# Autodesk Inventor assembly: Ansamblu
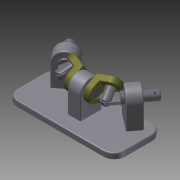
[picture p0: Inventor's stored thumbnail of the model, 180x180]
Saved by Autodesk Inventor 2011 SP2 (Build 150309200, 309)
## iProperties
Created: 2023-03-20
Part Number: Ansamblu
Document SubType Name: Assembly
Designer: utilizator
Author: utilizator
## Documents named in this file (7)
- D:\Studenti\Donisan Enya 1322b\Lab 4\Ansamblu.iam
- D:\Studenti\Donisan Enya 1322b\Lab 4\Placa.ipt
- D:\Studenti\Donisan Enya 1322b\Lab 4\Lagar.ipt
- D:\Studenti\Donisan Enya 1322b\Lab 4\Levier.ipt
- D:\Studenti\Donisan Enya 1322b\Lab 4\Furca.ipt
- D:\Studenti\Donisan Enya 1322b\Lab 4\Arbore.ipt
- D:\Studenti\Donisan Enya 1322b\Lab 4\Ax.ipt
## Components (11 placed, 6 different names)
1. Placa:1 — Mate:1, Mate:2, Mate:3, Mate:4, Mate:5, Angle:1, Angle:2
2. Lagar:1 — Mate:1, Angle:1, Insert:6, Mate:6, Mate:9
3. Lagar:2 — Mate:2, Mate:4, Mate:5, Insert:1, Insert:2
4. Lagar:3 — Mate:3, Angle:2, Insert:7, Mate:7, Mate:8
5. Levier:1 — Insert:1, Insert:3, Insert:4, Angle:3, Mate:6, Mate:9
6. Levier:2 — Insert:2, Insert:5, Angle:3, Mate:7, Mate:8
7. Furca:1 — Insert:4, Angle:4
8. Furca:2 — Insert:5, Angle:5
9. Arbore:1 — Insert:6, Angle:4
10. Arbore:2 — Insert:7, Angle:5
11. Ax:1 — Insert:3
## Relationships (21: Mate 9, Insert 7, Angle 5)
- Mate:1: Placa:1 ↔ Lagar:1
- Mate:2: Placa:1 ↔ Lagar:2
- Mate:3: Placa:1 ↔ Lagar:3
- Mate:4: Placa:1 ↔ Lagar:2
- Mate:5: Placa:1 ↔ Lagar:2
- Angle:1 (37.3 deg): Placa:1 ↔ Lagar:1
- Angle:2 (37.3 deg): Placa:1 ↔ Lagar:3
- Insert:1: Lagar:2 ↔ Levier:1
- Insert:2: Lagar:2 ↔ Levier:2
- Insert:3: Levier:1 ↔ Ax:1
- Insert:4: Levier:1 ↔ Furca:1
- Insert:5: Levier:2 ↔ Furca:2
- Angle:3 (0 deg): Levier:1 ↔ Levier:2
- Insert:6: Lagar:1 ↔ Arbore:1
- Insert:7: Lagar:3 ↔ Arbore:2
- Angle:4 (0 deg): Furca:1 ↔ Arbore:1
- Angle:5 (0 deg): Furca:2 ↔ Arbore:2
- Mate:6: Lagar:1 ↔ Levier:1
- Mate:7: Lagar:3 ↔ Levier:2
- Mate:8 (23 mm): Lagar:3 ↔ Levier:2
- Mate:9 (23 mm): Lagar:1 ↔ Levier:1
